# Autodesk Inventor assembly: hinge main
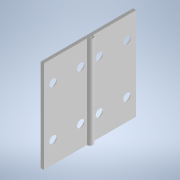
[picture p0: Inventor's stored thumbnail of the model, 180x180]
Saved by Autodesk Inventor 2021 (Build 250183000, 183)
## iProperties
Created: 2021-01-11
Part Number: hinge main
Document SubType Name: Assembly
Designer: Adam
Author: Adam
## Documents named in this file (4)
- C:\Users\Adam\Desktop\hinge main.iam
- C:\Users\Adam\Desktop\hinge 1.ipt
- C:\Users\Adam\Desktop\hinge 2.ipt
- C:\Users\Adam\Desktop\pret xd.ipt
## Components (3 placed, 3 different names)
1. hinge 1:1 — Kątowe:1, Wstawiające:1, Zestawiające:1
2. hinge 2:1 — Kątowe:1, Wstawiające:1, Wstawiające:2
3. pret xd:1 — Zestawiające:1, Wstawiające:2
## Relationships (4: Insert 2, Angle 1, Mate 1)
- Kątowe:1 [Angle] (0 deg): hinge 1:1 ↔ hinge 2:1
- Wstawiające:1 [Insert]: hinge 1:1 ↔ hinge 2:1
- Zestawiające:1 [Mate]: hinge 1:1 ↔ pret xd:1
- Wstawiające:2 [Insert]: hinge 2:1 ↔ pret xd:1
